# Autodesk Inventor assembly: Full_ServoBlock
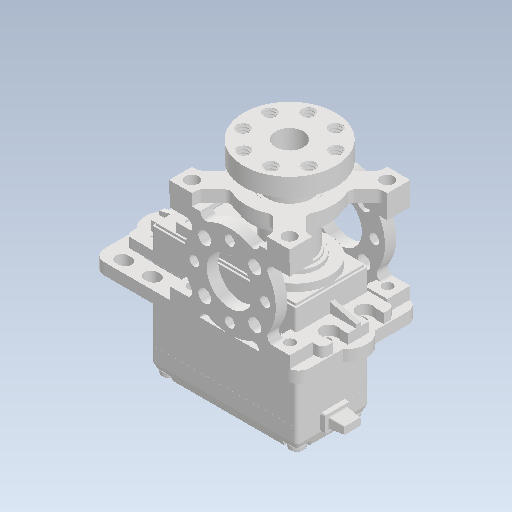
[picture p0: Inventor's stored thumbnail of the model, 512x512]
Saved by Autodesk Inventor 2020 (Build 240168000, 168)
## iProperties
Created: 2020-11-26
Part Number: Full_ServoBlock
Document SubType Name: Assembly
Designer: tdmp4
Author: tdmp4
## Documents named in this file (6)
- C:\Users\tdmp4\Documents\GitHub\CAD-2021-Ultimate_Goal\ServoCity\Full_ServoBlock.iam
- C:\Users\tdmp4\Documents\GitHub\CAD-2021-Ultimate_Goal\ServoCity\535118 assembly.ipt
- C:\Users\tdmp4\Documents\GitHub\CAD-2021-Ultimate_Goal\ServoCity\525123.ipt
- C:\Users\tdmp4\Documents\GitHub\CAD-2021-Ultimate_Goal\ServoCity\545420.ipt
- C:\Users\tdmp4\Documents\GitHub\CAD-2021-Ultimate_Goal\ServoCity\575112.ipt
- C:\Users\tdmp4\Documents\GitHub\CAD-2021-Ultimate_Goal\ServoCity\2000-0025-0002.ipt
## Components (6 placed, 5 different names)
1. 535118 assembly:1 — Mate:3, Flush:5, Flush:6, Mate:8
2. 525123:1 — Mate:7, Mate:8
3. 545420:1 — Mate:1, Flush:1, Flush:2, Flush:6
4. 545420:2 — Mate:2, Flush:3, Flush:4, Mate:3, Flush:5
5. 575112:1 — Mate:1, Flush:1, Flush:2, Mate:2, Flush:3, Flush:4, Mate:4, Mate:5, Mate:6
6. 2000-0025-0002:1 — Mate:4, Mate:5, Mate:6, Mate:7
## Relationships (14: Mate 8, Flush 6)
- Mate:1: 545420:1 ↔ 575112:1
- Flush:1 (2.54 mm): 545420:1 ↔ 575112:1
- Flush:2: 545420:1 ↔ 575112:1
- Mate:2: 545420:2 ↔ 575112:1
- Flush:3 (2.54 mm): 545420:2 ↔ 575112:1
- Flush:4: 545420:2 ↔ 575112:1
- Mate:3: 535118 assembly:1 ↔ 545420:2
- Flush:5: 535118 assembly:1 ↔ 545420:2
- Flush:6: 535118 assembly:1 ↔ 545420:1
- Mate:4: 575112:1 ↔ 2000-0025-0002:1
- Mate:5: 575112:1 ↔ 2000-0025-0002:1
- Mate:6: 575112:1 ↔ 2000-0025-0002:1
- Mate:7: 525123:1 ↔ 2000-0025-0002:1
- Mate:8: 535118 assembly:1 ↔ 525123:1
